# Autodesk Inventor assembly: 사이클로이드 기어 000.ipt
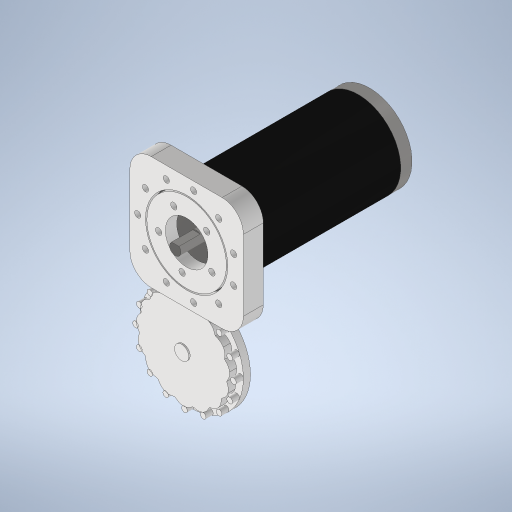
[picture p0: Inventor's stored thumbnail of the model, 512x512]
Saved by Autodesk Inventor 2023 (Build 270158000, 158)
## iProperties
Created: 2022-06-19
Part Number: 사이클로이드 기어 000.ipt
Document SubType Name: Assembly
Designer: fly01
Author: fly01
## Documents named in this file (8)
- C:\Users\fly01\Desktop\베이맥스\설계\설계 테스트\사이클로이드 기어 000.ipt.iam
- C:\Users\fly01\Desktop\베이맥스\설계\설계 테스트\사이클로이드 기어 001.ipt
- C:\Users\fly01\Desktop\베이맥스\설계\설계 테스트\사이클로이드 기어 002.ipt
- C:\Users\fly01\Desktop\베이맥스\설계\설계 테스트\사이클로이드 기어 003.ipt
- C:\Users\fly01\Desktop\베이맥스\설계\설계 테스트\사이클로이드 기어 하우징.ipt
- C:\Users\fly01\Desktop\베이맥스\설계\범용 부품\중형 모터 MB60080-2430 DC24V.ipt
- C:\Users\fly01\Desktop\베이맥스\설계\범용 부품\6810베어링.ipt
- C:\Users\fly01\Desktop\베이맥스\설계\설계 테스트\사이클로이드 기어 축 연결 하우징.ipt
## Components (7 placed, 7 different names)
1. 사이클로이드 기어 001:1 — 삽입:1
2. 사이클로이드 기어 002:1 — 삽입:2
3. 사이클로이드 기어 003:1 — 삽입:1, 삽입:2
4. 사이클로이드 기어 하우징:1 — 삽입:3, 삽입:4, 삽입:5
5. 중형 모터 MB60080-2430 DC24V:1 — 삽입:4, 삽입:5
6. 6810베어링:1 — 삽입:3, 삽입:6
7. 사이클로이드 기어 축 연결 하우징:1 — 삽입:6
## Relationships (6: Insert 6)
- 삽입:1 [Insert]: 사이클로이드 기어 001:1 ↔ 사이클로이드 기어 003:1
- 삽입:2 [Insert]: 사이클로이드 기어 002:1 ↔ 사이클로이드 기어 003:1
- 삽입:3 [Insert]: 사이클로이드 기어 하우징:1 ↔ 6810베어링:1
- 삽입:4 [Insert]: 사이클로이드 기어 하우징:1 ↔ 중형 모터 MB60080-2430 DC24V:1
- 삽입:5 [Insert]: 사이클로이드 기어 하우징:1 ↔ 중형 모터 MB60080-2430 DC24V:1
- 삽입:6 [Insert]: 6810베어링:1 ↔ 사이클로이드 기어 축 연결 하우징:1
